# Autodesk Inventor assembly: ASSEMBLY
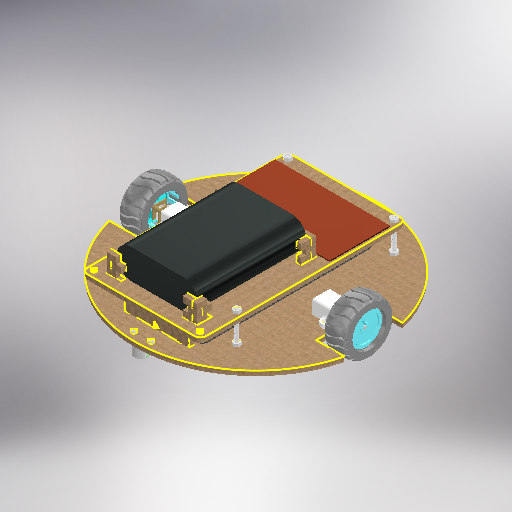
[picture p0: Inventor's stored thumbnail of the model, 512x512]
Saved by Autodesk Inventor 2025 (Build 290162000, 162)
## iProperties
Created: 2024-09-26
Part Number: ASSEMBLY
Document SubType Name: Assembly
Designer: DANIEL
Checked By: FERNANDO
Engr Approved By: ANTONIO
Stock Number: 1
Author: DANIEL
Title: ASSEMBLY
## Documents named in this file (16)
- C:\Users\DANIEL\Documents\EIA\Semestres\08\RoboticaIndustrial\labs\06\DIFFCAR_CAD\ASSEMBLY.iam
- C:\Users\DANIEL\Documents\EIA\Semestres\08\RoboticaIndustrial\labs\06\DIFFCAR_CAD\base.ipt
- C:\Users\DANIEL\Documents\EIA\Semestres\08\RoboticaIndustrial\labs\06\DIFFCAR_CAD\step_cadmodels\N20 DC MOTOR\N20 DC MOTOR.ipt
- C:\Users\DANIEL\Documents\EIA\Semestres\08\RoboticaIndustrial\labs\06\DIFFCAR_CAD\step_cadmodels\N20_Bracket_Extended_Pololu\N20_Bracket_Extended_Pololu.ipt
- C:\Users\DANIEL\Documents\EIA\Semestres\08\RoboticaIndustrial\labs\06\DIFFCAR_CAD\step_cadmodels\RC wheel\RC wheel.ipt
- C:\Users\DANIEL\Documents\EIA\Semestres\08\RoboticaIndustrial\labs\06\DIFFCAR_CAD\step_cadmodels\caster\caster.ipt
- C:\Users\DANIEL\Documents\EIA\Semestres\08\RoboticaIndustrial\labs\06\DIFFCAR_CAD\PI4_housing.ipt
- C:\Users\DANIEL\Documents\EIA\Semestres\08\RoboticaIndustrial\labs\06\DIFFCAR_CAD\powerbank.ipt
- C:\Users\DANIEL\Documents\EIA\Semestres\08\RoboticaIndustrial\labs\06\DIFFCAR_CAD\bakelite.ipt
- C:\Users\DANIEL\Documents\EIA\Semestres\08\RoboticaIndustrial\labs\06\DIFFCAR_CAD\step_cadmodels\screwM3X30\screwM3X30.ipt
- C:\Users\DANIEL\Documents\EIA\Semestres\08\RoboticaIndustrial\labs\06\DIFFCAR_CAD\step_cadmodels\nutM3\nutM3.ipt
- C:\Users\DANIEL\Documents\EIA\Semestres\08\RoboticaIndustrial\labs\06\DIFFCAR_CAD\upper_plate.ipt
- C:\Users\DANIEL\Documents\EIA\Semestres\08\RoboticaIndustrial\labs\06\DIFFCAR_CAD\wall1.ipt
- C:\Users\DANIEL\Documents\EIA\Semestres\08\RoboticaIndustrial\labs\06\DIFFCAR_CAD\corner.iam
- C:\Users\DANIEL\Documents\EIA\Semestres\08\RoboticaIndustrial\labs\06\DIFFCAR_CAD\step_cadmodels\screwM2X10\screwM2X10.ipt
- C:\Users\DANIEL\Documents\EIA\Semestres\08\RoboticaIndustrial\labs\06\DIFFCAR_CAD\step_cadmodels\nutM2\nutM2.ipt
## Components (46 placed, 15 different names)
1. base:1 — Mate:2, Mate:4, Mate:5, Mate:6, Mate:7, Mate:8, Mate:10, Tangent:1, Mate:11, Mate:12, Mate:13, Mate:15, Mate:17, Mate:18, Mate:19, Mate:20, Insert:7, Insert:8, Mate:23, Mate:24, Mate:25, Mate:26, Mate:27, Mate:28, Insert:9, Insert:10, Insert:11, Insert:16, Insert:17, Insert:20, Insert:21, Insert:22, Insert:23
2. N20 DC MOTOR:1 — Mate:3, Flush:2, Mate:4, Mate:22, Tangent:3
3. N20 DC MOTOR:2 — Mate:1, Flush:1, Mate:2, Mate:21, Tangent:2
4. N20_Bracket_Extended_Pololu:1 — Mate:7, Angle:5, Flush:4, Mate:21, Tangent:2, Insert:24, Insert:25
5. N20_Bracket_Extended_Pololu:2 — Mate:6, Insert:7, Insert:8, Mate:22, Tangent:3, Insert:26, Insert:27
6. RC wheel:1 — Mate:1, Flush:1, Angle:2
7. RC wheel:2 — Mate:3, Flush:2, Angle:1
8. caster:1 — Mate:5, Tangent:1, Flush:3, Insert:18, Insert:19
9. powerbank:1 — Mate:8, Angle:3
10. PI4_housing:1 — Mate:9, Angle:4
11. bakelite:1 — Mate:16
12. screwM3X30:1 — Mate:10, Mate:20, Insert:2
13. screwM3X30:2 — Mate:13, Mate:14, Mate:17, Insert:1
14. screwM3X30:3 — Mate:11, Mate:19, Insert:3
15. screwM3X30:4 — Mate:12, Mate:18, Insert:4
16. nutM3:1 — Mate:14, Mate:15
17. nutM3:2 — Insert:3
18. nutM3:3 — Insert:2, Insert:6
19. nutM3:4 — Insert:1
20. upper_plate:1 — Mate:9, Mate:16, Insert:5, Insert:6, Mate:29, Mate:30, Mate:31, Mate:32, Mate:33, Mate:34, Mate:35, Mate:36, Flush:5, Mate:37, Mate:38, Mate:39, Flush:6, Mate:40, Insert:12, Insert:13, Insert:14, Insert:15
21. nutM3:5 — Insert:4, Insert:5
22. wall1:1 — Mate:23, Mate:24, Mate:25
23. wall1:2 — Mate:26, Mate:27, Mate:28
24. corner:1 [sub-assembly] — Mate:29, Mate:30, Mate:31
25. corner:2 [sub-assembly] — Mate:37, Mate:38, Mate:39, Flush:6, Mate:40
26. corner:3 [sub-assembly] — Mate:35, Mate:36, Flush:5
27. corner:4 [sub-assembly] — Mate:32, Mate:33, Mate:34
28. nutM3:6 — Insert:9
29. nutM3:7 — Insert:10
30. nutM3:8 — Insert:12
31. nutM3:9 — Insert:13
32. nutM3:10 — Insert:11
33. nutM3:11 — Insert:14
34. nutM3:12 — Insert:15
35. screwM2X10:1 — Insert:16
36. screwM2X10:2 — Insert:17
37. screwM2X10:3 — Insert:23
38. screwM2X10:4 — Insert:22
39. screwM2X10:5 — Insert:21
40. screwM2X10:6 — Insert:20
41. nutM2:1 — Insert:18
42. nutM2:2 — Insert:19
43. nutM2:3 — Insert:24
44. nutM2:4 — Insert:25
45. nutM2:5 — Insert:27
46. nutM2:6 — Insert:26
## Relationships (81: Mate 40, Insert 27, Flush 6, Angle 5, Tangent 3)
- Mate:1: N20 DC MOTOR:2 ↔ RC wheel:1
- Flush:1: N20 DC MOTOR:2 ↔ RC wheel:1
- Mate:2: base:1 ↔ N20 DC MOTOR:2
- Mate:3: N20 DC MOTOR:1 ↔ RC wheel:2
- Flush:2: N20 DC MOTOR:1 ↔ RC wheel:2
- Mate:4: base:1 ↔ N20 DC MOTOR:1
- Mate:5: base:1 ↔ caster:1
- Mate:6: base:1 ↔ N20_Bracket_Extended_Pololu:2
- Mate:7: base:1 ↔ N20_Bracket_Extended_Pololu:1
- Angle:1 (180 deg): RC wheel:2
- Angle:2 (0 deg): RC wheel:1
- Mate:8: base:1 ↔ powerbank:1
- Mate:9: PI4_housing:1 ↔ upper_plate:1
- Angle:3 (0 deg): powerbank:1
- Mate:10: base:1 ↔ screwM3X30:1
- Tangent:1: base:1 ↔ caster:1
- Flush:3: caster:1
- Mate:11: base:1 ↔ screwM3X30:3
- Mate:12: base:1 ↔ screwM3X30:4
- Mate:13: base:1 ↔ screwM3X30:2
- Mate:14: screwM3X30:2 ↔ nutM3:1
- Mate:15: base:1 ↔ nutM3:1
- Angle:4 (90 deg): PI4_housing:1
- Mate:16: bakelite:1 ↔ upper_plate:1
- Mate:17: base:1 ↔ screwM3X30:2
- Mate:18: base:1 ↔ screwM3X30:4
- Mate:19: base:1 ↔ screwM3X30:3
- Mate:20: base:1 ↔ screwM3X30:1
- Insert:1: screwM3X30:2 ↔ nutM3:4
- Insert:2: screwM3X30:1 ↔ nutM3:3
- Insert:3: screwM3X30:3 ↔ nutM3:2
- Insert:4: screwM3X30:4 ↔ nutM3:5
- Insert:5: upper_plate:1 ↔ nutM3:5
- Insert:6: nutM3:3 ↔ upper_plate:1
- Angle:5 (180 deg): N20_Bracket_Extended_Pololu:1
- Flush:4: N20_Bracket_Extended_Pololu:1
- Mate:21: N20 DC MOTOR:2 ↔ N20_Bracket_Extended_Pololu:1
- Tangent:2: N20 DC MOTOR:2 ↔ N20_Bracket_Extended_Pololu:1
- Insert:7: base:1 ↔ N20_Bracket_Extended_Pololu:2
- Insert:8: base:1 ↔ N20_Bracket_Extended_Pololu:2
- Mate:22: N20 DC MOTOR:1 ↔ N20_Bracket_Extended_Pololu:2
- Tangent:3: N20 DC MOTOR:1 ↔ N20_Bracket_Extended_Pololu:2
- Mate:23: base:1 ↔ wall1:1
- Mate:24: base:1 ↔ wall1:1
- Mate:25: base:1 ↔ wall1:1
- Mate:26: base:1 ↔ wall1:2
- Mate:27: base:1 ↔ wall1:2
- Mate:28: base:1 ↔ wall1:2
- Mate:29: upper_plate:1 ↔ corner:1
- Mate:30: upper_plate:1 ↔ corner:1
- Mate:31: upper_plate:1 ↔ corner:1
- Mate:32: upper_plate:1 ↔ corner:4
- Mate:33: upper_plate:1 ↔ corner:4
- Mate:34: upper_plate:1 ↔ corner:4
- Mate:35: upper_plate:1 ↔ corner:3
- Mate:36: upper_plate:1 ↔ corner:3
- Flush:5: upper_plate:1 ↔ corner:3
- Mate:37: upper_plate:1 ↔ corner:2
- Mate:38: upper_plate:1 ↔ corner:2
- Mate:39: upper_plate:1 ↔ corner:2
- Flush:6: upper_plate:1 ↔ corner:2
- Mate:40: upper_plate:1 ↔ corner:2
- Insert:9: base:1 ↔ nutM3:6
- Insert:10: base:1 ↔ nutM3:7
- Insert:11: base:1 ↔ nutM3:10
- Insert:12: upper_plate:1 ↔ nutM3:8
- Insert:13: upper_plate:1 ↔ nutM3:9
- Insert:14: upper_plate:1 ↔ nutM3:11
- Insert:15: upper_plate:1 ↔ nutM3:12
- Insert:16: base:1 ↔ screwM2X10:1
- Insert:17: base:1 ↔ screwM2X10:2
- Insert:18: caster:1 ↔ nutM2:1
- Insert:19: caster:1 ↔ nutM2:2
- Insert:20: base:1 ↔ screwM2X10:6
- Insert:21: base:1 ↔ screwM2X10:5
- Insert:22: base:1 ↔ screwM2X10:4
- Insert:23: base:1 ↔ screwM2X10:3
- Insert:24: N20_Bracket_Extended_Pololu:1 ↔ nutM2:3
- Insert:25: N20_Bracket_Extended_Pololu:1 ↔ nutM2:4
- Insert:26: N20_Bracket_Extended_Pololu:2 ↔ nutM2:6
- Insert:27: N20_Bracket_Extended_Pololu:2 ↔ nutM2:5
